# Autodesk Inventor assembly: Elevator
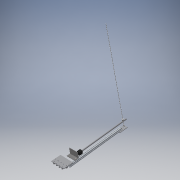
[picture p0: Inventor's stored thumbnail of the model, 180x180]
Saved by Autodesk Inventor 2017 (Build 210142000, 142)
## iProperties
Created: 2016-12-12
Part Number: Elevator
Document SubType Name: Assembly
Designer: umr
Mass: 4376.08 g
Surface Area: 10170.9 cm^2
Volume: 1553.17 cm^3
Density: 2.81752 g/cm^3
Author: umr
## Documents named in this file (14)
- D:\SeniorProject\Models2\Gantry\GantryDown.iam
- D:\SeniorProject\Models2\Gantry\Gantry Plate.ipt
- D:\SeniorProject\Models2\Gantry\M5 Screw with Tee Nut.iam
- D:\SeniorProject\Models2\Gantry\Solid Wheel with Eccentric Spacer Assembly.iam
- D:\SeniorProject\Models2\Gantry\L_Fixer.ipt
- D:\SeniorProject\Models2\Gantry\ScrewDriver.ipt
- D:\SeniorProject\Models2\Gantry\Motor.ipt
- D:\SeniorProject\Models2\Gantry\Motor Mount Plate.ipt
- D:\SeniorProject\Models2\Gantry\Driveshaft.ipt
- D:\SeniorProject\Models2\Gantry\5mm x 5mm Flexible Coupling.ipt
- D:\SeniorProject\Models2\Gantry\GT2 20 Tooth Pulley.ipt
- D:\SeniorProject\Models2\Gantry\Elevator Track30x30.ipt
- D:\SeniorProject\Models2\GanrtyPlatev2.ipt
- D:\SeniorProject\Models2\MotorPlate.ipt
## Components (31 placed, 13 different names)
1. Gantry Plate:1 — Mate:3, Mate:7, Mate:9, Mate:13, Mate:14, Mate:17
2. M5 Screw with Tee Nut:2 [sub-assembly] — Mate:3, Mate:14, Mate:112
3. M5 Screw with Tee Nut:6 [sub-assembly] — Mate:7, Mate:13, Mate:118
4. M5 Screw with Tee Nut:8 [sub-assembly] — Mate:9, Mate:17, Mate:120
5. L_Fixer:1 — Mate:113, Flush:1, Mate:117, Mate:126
6. M5 Screw with Tee Nut:10 [sub-assembly] — Mate:117, Mate:126
7. ScrewDriver:1 — Mate:72, Mate:73
8. Motor:1 — Mate:72, Mate:73
9. Motor Mount Plate:1 — Mate:88, Mate:89, Mate:90, Mate:91
10. M5 Screw with Tee Nut:15 [sub-assembly] — Mate:89, Mate:91
11. M5 Screw with Tee Nut:16 [sub-assembly] — Mate:90
12. M5 Screw with Tee Nut:17 [sub-assembly] — Mate:88
13. Motor:2 — Mate:140, Mate:141, Mate:145
14. 5mm x 5mm Flexible Coupling:1 — Mate:97
15. Driveshaft:1 — Mate:97, Mate:145, Mate:146, Mate:147
16. GT2 20 Tooth Pulley:1 — Mate:147
17. Elevator Track30x30:1 — Mate:112, Mate:113, Flush:1, Mate:121, Mate:134, Mate:135, Mate:136
18. GanrtyPlatev2:1 — Mate:118, Mate:120, Mate:121, Mate:122, Mate:123, Mate:124, Mate:125
19. M5 Screw with Tee Nut:18 [sub-assembly] — Mate:136, Mate:143
20. M5 Screw with Tee Nut:19 [sub-assembly] — Mate:134, Mate:135, Mate:142
21. M5 Screw with Tee Nut:20 [sub-assembly] — Mate:144
22. MotorPlate:1 — Mate:140, Mate:141, Mate:142, Mate:143, Mate:144, Mate:146
23. Solid Wheel with Eccentric Spacer Assembly:2 [sub-assembly] — Mate:122, Mate:123
24. Solid Wheel with Eccentric Spacer Assembly:3 [sub-assembly]
25. Solid Wheel with Eccentric Spacer Assembly:4 [sub-assembly]
26. Solid Wheel with Eccentric Spacer Assembly:5 [sub-assembly]
27. Solid Wheel with Eccentric Spacer Assembly:6 [sub-assembly]
28. Solid Wheel with Eccentric Spacer Assembly:7 [sub-assembly] — Mate:124, Mate:125
29. Solid Wheel with Eccentric Spacer Assembly:8 [sub-assembly]
30. Solid Wheel with Eccentric Spacer Assembly:9 [sub-assembly]
31. Solid Wheel with Eccentric Spacer Assembly:10 [sub-assembly]
## Component patterns: (5 elements, first: Solid Wheel with Eccentric Spacer Assembly:2), (4 elements, first: Solid Wheel with Eccentric Spacer Assembly:7)
## Relationships (36: Mate 35, Flush 1)
- Mate:3: Gantry Plate:1 ↔ M5 Screw with Tee Nut:2
- Mate:7: Gantry Plate:1 ↔ M5 Screw with Tee Nut:6
- Mate:9: Gantry Plate:1 ↔ M5 Screw with Tee Nut:8
- Mate:13: Gantry Plate:1 ↔ M5 Screw with Tee Nut:6
- Mate:14: Gantry Plate:1 ↔ M5 Screw with Tee Nut:2
- Mate:17: Gantry Plate:1 ↔ M5 Screw with Tee Nut:8
- Mate:72: ScrewDriver:1 ↔ Motor:1
- Mate:73: ScrewDriver:1 ↔ Motor:1
- Mate:88: Motor Mount Plate:1 ↔ M5 Screw with Tee Nut:17
- Mate:89: Motor Mount Plate:1 ↔ M5 Screw with Tee Nut:15
- Mate:90: Motor Mount Plate:1 ↔ M5 Screw with Tee Nut:16
- Mate:91: Motor Mount Plate:1 ↔ M5 Screw with Tee Nut:15
- Mate:97: 5mm x 5mm Flexible Coupling:1 ↔ Driveshaft:1
- Mate:112: M5 Screw with Tee Nut:2 ↔ Elevator Track30x30:1
- Mate:113: L_Fixer:1 ↔ Elevator Track30x30:1
- Flush:1: L_Fixer:1 ↔ Elevator Track30x30:1
- Mate:117: L_Fixer:1 ↔ M5 Screw with Tee Nut:10
- Mate:118: M5 Screw with Tee Nut:6 ↔ GanrtyPlatev2:1
- Mate:120: M5 Screw with Tee Nut:8 ↔ GanrtyPlatev2:1
- Mate:121: Elevator Track30x30:1 ↔ GanrtyPlatev2:1
- Mate:122: GanrtyPlatev2:1 ↔ Solid Wheel with Eccentric Spacer Assembly:2
- Mate:123: GanrtyPlatev2:1 ↔ Solid Wheel with Eccentric Spacer Assembly:2
- Mate:124: GanrtyPlatev2:1 ↔ Solid Wheel with Eccentric Spacer Assembly:7
- Mate:125: GanrtyPlatev2:1 ↔ Solid Wheel with Eccentric Spacer Assembly:7
- Mate:126: L_Fixer:1 ↔ M5 Screw with Tee Nut:10
- Mate:134: Elevator Track30x30:1 ↔ M5 Screw with Tee Nut:19
- Mate:135: Elevator Track30x30:1 ↔ M5 Screw with Tee Nut:19
- Mate:136: Elevator Track30x30:1 ↔ M5 Screw with Tee Nut:18
- Mate:140: Motor:2 ↔ MotorPlate:1
- Mate:141: Motor:2 ↔ MotorPlate:1
- Mate:142: M5 Screw with Tee Nut:19 ↔ MotorPlate:1
- Mate:143: M5 Screw with Tee Nut:18 ↔ MotorPlate:1
- Mate:144: M5 Screw with Tee Nut:20 ↔ MotorPlate:1
- Mate:145: Motor:2 ↔ Driveshaft:1
- Mate:146: Driveshaft:1 ↔ MotorPlate:1
- Mate:147: Driveshaft:1 ↔ GT2 20 Tooth Pulley:1
